# Autodesk Inventor assembly: A2017_T3_01
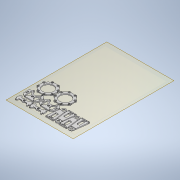
[picture p0: Inventor's stored thumbnail of the model, 180x180]
Saved by Autodesk Inventor 2020 (Build 240168000, 168)
## iProperties
Created: 2021-08-27
Part Number: A2017_T3_01
Document SubType Name: Assembly
Designer: Masato
Author: Masato
## Documents named in this file (6)
- C:\Users\naoki\Documents\Inventor\CitBrains\git_clone\OpenPlatform4_0\CAM\A2017_T3\OpenPlatform_ver3_0\cam\A2017_T3_01.iam
- C:\Users\naoki\Documents\Inventor\CitBrains\git_clone\OpenPlatform4_0\CAM\A2017_T3\OpenPlatform_ver3_0\cam\Disposable_Board.ipt
- C:\Users\naoki\Documents\Inventor\CitBrains\git_clone\OpenPlatform4_0\CAM\A2017_T3\OpenPlatform_ver3_0\LowerBody\Ankle\Ankle_front_frame.ipt
- C:\Users\naoki\Documents\Inventor\CitBrains\git_clone\OpenPlatform4_0\CAM\A2017_T3\OpenPlatform_ver3_0\LowerBody\Leg_joit\Leg_joint_roll_front_frame.ipt
- C:\Users\naoki\Documents\Inventor\CitBrains\git_clone\OpenPlatform4_0\CAM\A2017_T3\OpenPlatform_ver3_0\LowerBody\Leg_joit\Leg_joint_slider_frame.ipt
- C:\Users\naoki\Documents\Inventor\CitBrains\git_clone\OpenPlatform4_0\CAM\A2017_T3\OpenPlatform_ver3_0\UpperBody\Trunk\Outer_flange.ipt
## Components (11 placed, 5 different names)
1. Disposable_Board:1 — メイト:2, メイト:1, フラッシュ:1, フラッシュ:2, フラッシュ:3, フラッシュ:4, フラッシュ:5, 正接:2, フラッシュ:6, 正接:4, 正接:5
2. Ankle_front_frame:1 — メイト:7, フラッシュ:3, フラッシュ:4, 正接:1
3. Ankle_front_frame:2
4. Leg_joint_roll_front_frame:1 — メイト:6, フラッシュ:5, 正接:1, 正接:6
5. Leg_joint_roll_front_frame:2 — 正接:3
6. Leg_joint_slider_frame:2 — メイト:8, フラッシュ:6, 正接:3, メイト:9
7. Leg_joint_slider_frame:1 — メイト:4, メイト:8, 正接:2
8. Leg_joint_slider_frame:3
9. Leg_joint_slider_frame:4
10. Outer_flange:1 — メイト:5, 正接:4, 正接:5, 正接:6
11. Outer_flange:2
## Component patterns: (2 elements, first: Ankle_front_frame:1), (2 elements, first: Leg_joint_roll_front_frame:1), (2 elements, first: Leg_joint_slider_frame:2 + Leg_joint_slider_frame:1), (2 elements, first: Outer_flange:1)
## Relationships (20: Mate 8, Flush 6, Tangent 6)
- メイト:2 [Mate]: Disposable_Board:1
- メイト:1 [Mate]: Disposable_Board:1
- フラッシュ:1 [Flush]: Disposable_Board:1
- フラッシュ:2 [Flush]: Disposable_Board:1
- メイト:4 [Mate]: Leg_joint_slider_frame:1
- メイト:5 [Mate]: Outer_flange:1
- メイト:6 [Mate]: Leg_joint_roll_front_frame:1
- メイト:7 [Mate]: Ankle_front_frame:1
- フラッシュ:3 [Flush] (2 mm): Disposable_Board:1 ↔ Ankle_front_frame:1
- フラッシュ:4 [Flush] (1 mm): Disposable_Board:1 ↔ Ankle_front_frame:1
- フラッシュ:5 [Flush] (1 mm): Disposable_Board:1 ↔ Leg_joint_roll_front_frame:1
- 正接:1 [Tangent] (2.5 mm): Ankle_front_frame:1 ↔ Leg_joint_roll_front_frame:1
- メイト:8 [Mate] (2.5 mm): Leg_joint_slider_frame:2 ↔ Leg_joint_slider_frame:1
- 正接:2 [Tangent] (2 mm): Disposable_Board:1 ↔ Leg_joint_slider_frame:1
- フラッシュ:6 [Flush] (2 mm): Disposable_Board:1 ↔ Leg_joint_slider_frame:2
- 正接:3 [Tangent] (2.5 mm): Leg_joint_roll_front_frame:2 ↔ Leg_joint_slider_frame:2
- 正接:4 [Tangent] (2 mm): Disposable_Board:1 ↔ Outer_flange:1
- 正接:5 [Tangent] (2 mm): Disposable_Board:1 ↔ Outer_flange:1
- 正接:6 [Tangent] (2.5 mm): Leg_joint_roll_front_frame:1 ↔ Outer_flange:1
- メイト:9 [Mate]: Leg_joint_slider_frame:2
